# Autodesk Inventor assembly: s-assy-link4+5+gripper
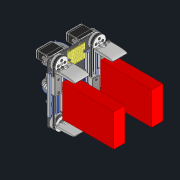
[picture p0: Inventor's stored thumbnail of the model, 180x180]
Saved by Autodesk Inventor 2021 (Build 250183000, 183)
## iProperties
Created: 2021-08-13
Part Number: s-assy-link4+5+gripper
Document SubType Name: Assembly
Designer: yuta0
Mass: 948.793 g
Surface Area: 3076.1 cm^2
Volume: 422.495 cm^3
Density: 2.24569 g/cm^3
Author: yuta0
## Documents named in this file (5)
- C:\Users\yuta0\Documents\GitHub\catchrobo_hardware\assy-robot\s-assy-link4+5+gripper.iam
- C:\Users\yuta0\Documents\GitHub\catchrobo_hardware\assy-robot\s-assy-gripper.iam
- C:\Users\yuta0\Documents\GitHub\catchrobo_hardware\assy-robot\s-assy-link4.iam
- C:\Users\yuta0\Documents\GitHub\catchrobo_hardware\assy-robot\base7.ipt
- C:\Users\yuta0\Downloads\新しいフォルダー\bisco.ipt
## Components (5 placed, 4 different names)
1. s-assy-link4:1 [sub-assembly] — メイト:1, メイト:3, メイト:4
2. s-assy-gripper:1 [sub-assembly] — メイト:2, メイト:4, フラッシュ:2, メイト:5, メイト:6, メイト:7
3. base7:1 — メイト:1, フラッシュ:1, メイト:2, メイト:3
4. bisco:1 — フラッシュ:2, メイト:5, メイト:7
5. bisco:2
## Component patterns: (2 elements, first: bisco:1)
## Relationships (9: Mate 7, Flush 2)
- メイト:1 [Mate]: s-assy-link4:1 ↔ base7:1
- フラッシュ:1 [Flush]: base7:1
- メイト:2 [Mate]: s-assy-gripper:1 ↔ base7:1
- メイト:3 [Mate]: s-assy-link4:1 ↔ base7:1
- メイト:4 [Mate]: s-assy-link4:1 ↔ s-assy-gripper:1
- フラッシュ:2 [Flush] (5.5 mm): s-assy-gripper:1 ↔ bisco:1
- メイト:5 [Mate] (5 mm): s-assy-gripper:1 ↔ bisco:1
- メイト:6 [Mate]: s-assy-gripper:1
- メイト:7 [Mate] (17 mm): s-assy-gripper:1 ↔ bisco:1
